# Autodesk Inventor assembly: ankle_w_motor_fin1
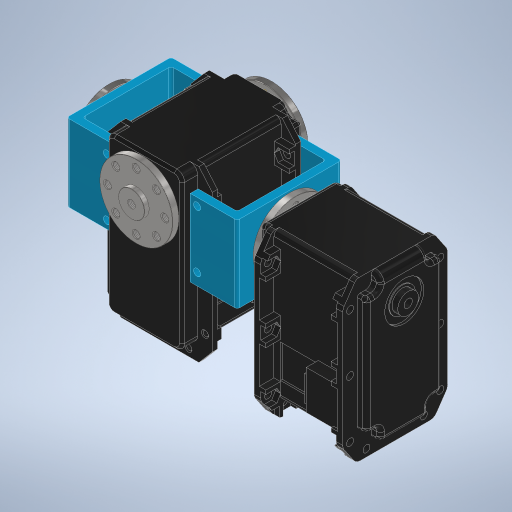
[picture p0: Inventor's stored thumbnail of the model, 512x512]
Saved by Autodesk Inventor 2024 (Build 280153000, 153)
## iProperties
Created: 2024-09-14
Part Number: ankle_w_motor_fin1
Document SubType Name: Assembly
Designer: jmha0
Author: jmha0
## Documents named in this file (8)
- C:\Users\jmha0\OneDrive\바탕 화면\19th_intern_hjm_fight_robot\Lower_Body\ankle_w_motor\ankle_w_motor_fin1.iam
- C:\Users\jmha0\OneDrive\바탕 화면\19th_intern_hjm_fight_robot\hardware\ROBOTIS(Inventor 2024 ver.)\다이나믹셀\MX-106T+idle.ipt.iam
- C:\Users\jmha0\OneDrive\바탕 화면\19th_intern_hjm_fight_robot\hardware\ROBOTIS(Inventor 2024 ver.)\혼\64-106Horn.ipt
- C:\Users\jmha0\OneDrive\바탕 화면\19th_intern_hjm_fight_robot\Lower_Body\ankle_w_motor\3D_ankle1.ipt
- C:\Users\jmha0\OneDrive\바탕 화면\19th_intern_hjm_fight_robot\Lower_Body\ankle_w_motor\3D_ankle2.ipt
- C:\Users\jmha0\OneDrive\바탕 화면\19th_intern_hjm_fight_robot\hardware\ROBOTIS(Inventor 2024 ver.)\아이들러\64아이들러.iam
- C:\Users\jmha0\OneDrive\바탕 화면\19th_intern_hjm_fight_robot\hardware\ROBOTIS(Inventor 2024 ver.)\다이나믹셀\MX-64T.ipt
- MX-106T+idle.ipt
## Components (7 placed, 6 different names)
1. MX-106T+idle.ipt:1 [sub-assembly] — 삽입:1, 삽입:2, 삽입:3, 삽입:4, 삽입:5, 삽입:6, 삽입:7, 삽입:8, 삽입:9
2. 64-106Horn:1 — 삽입:1
3. 3D_ankle1:1 — 삽입:2, 삽입:3, 삽입:4, 삽입:5, 삽입:10
4. 3D_ankle2:1 — 삽입:6, 삽입:7, 삽입:8, 삽입:9, 삽입:12, 삽입:13, 삽입:14, 삽입:15
5. 64아이들러:1 [sub-assembly] — 삽입:10
6. MX-64T:1 — 삽입:11
7. 64-106Horn:2 — 삽입:11, 삽입:12, 삽입:13, 삽입:14, 삽입:15
## Relationships (15: Insert 15)
- 삽입:1 [Insert] (0.1 mm): MX-106T+idle.ipt:1 ↔ 64-106Horn:1
- 삽입:2 [Insert]: MX-106T+idle.ipt:1 ↔ 3D_ankle1:1
- 삽입:3 [Insert]: MX-106T+idle.ipt:1 ↔ 3D_ankle1:1
- 삽입:4 [Insert]: MX-106T+idle.ipt:1 ↔ 3D_ankle1:1
- 삽입:5 [Insert]: MX-106T+idle.ipt:1 ↔ 3D_ankle1:1
- 삽입:6 [Insert]: MX-106T+idle.ipt:1 ↔ 3D_ankle2:1
- 삽입:7 [Insert]: MX-106T+idle.ipt:1 ↔ 3D_ankle2:1
- 삽입:8 [Insert]: MX-106T+idle.ipt:1 ↔ 3D_ankle2:1
- 삽입:9 [Insert]: MX-106T+idle.ipt:1 ↔ 3D_ankle2:1
- 삽입:10 [Insert] (0.1 mm): 3D_ankle1:1 ↔ 64아이들러:1
- 삽입:11 [Insert] (0.1 mm): MX-64T:1 ↔ 64-106Horn:2
- 삽입:12 [Insert]: 3D_ankle2:1 ↔ 64-106Horn:2
- 삽입:13 [Insert]: 3D_ankle2:1 ↔ 64-106Horn:2
- 삽입:14 [Insert]: 3D_ankle2:1 ↔ 64-106Horn:2
- 삽입:15 [Insert]: 3D_ankle2:1 ↔ 64-106Horn:2
